# Autodesk Inventor assembly: magnet_ring_assembly
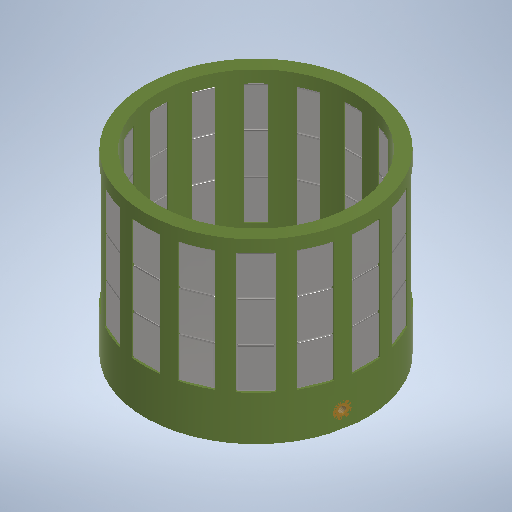
[picture p0: Inventor's stored thumbnail of the model, 512x512]
Saved by Autodesk Inventor 2025 (Build 290162000, 162)
## iProperties
Created: 2026-08-03
Part Number: magnet_ring_assembly
Document SubType Name: Assembly
Designer: zzapa
Author: zzapa
## Documents named in this file (4)
- C:\Users\zzapa\Desktop\Projekty\elektronika\engine-project\model\assemblies\magnet_ring_assembly.iam
- C:\Users\zzapa\Desktop\Projekty\elektronika\engine-project\model\parts\magnet_ring.ipt
- C:\Users\zzapa\Desktop\Projekty\elektronika\engine-project\model\parts\stator_magnet.ipt
- C:\Users\zzapa\Documents\Inventor\Content Center Files\R2025\pl-PL\GB 809-88 A\Nut GB 809 A M2 x 3.ipt
## Components (51 placed, 3 different names)
1. magnet_ring:1 — Zestawiające:1, Kątowe:1, Zestawiające:6, Równoległe:5, Zestawiające:7, Zestawiające:8, Równoległe:7, Zestawiające:9, Równoległe:8
2. Nut GB/T 809-1988 Type A M2x3:1 — Zestawiające:8, Równoległe:7
3. Nut GB/T 809-1988 Type A M2x3:2 — Zestawiające:9, Równoległe:8
4. stator_magnet:1 — Zestawiające:3, Równoległe:1, Równoległe:2, Zestawiające:6, Symetria:1, Symetria:2
5. stator_magnet:2 — Zestawiające:4, Równoległe:3, Równoległe:4, Symetria:1
6. stator_magnet:3 — Zestawiające:3, Równoległe:1, Zestawiające:4, Równoległe:2, Równoległe:3, Równoległe:4, Zestawiające:7, Symetria:2
7. stator_magnet:4
8. stator_magnet:5
9. stator_magnet:6
10. stator_magnet:7
11. stator_magnet:8
12. stator_magnet:9
13. stator_magnet:10
14. stator_magnet:11
15. stator_magnet:12
16. stator_magnet:13
17. stator_magnet:14
18. stator_magnet:15
19. stator_magnet:16
20. stator_magnet:17
21. stator_magnet:18
22. stator_magnet:19
23. stator_magnet:20
24. stator_magnet:21
25. stator_magnet:22
26. stator_magnet:23
27. stator_magnet:24 — Symetria:3
28. stator_magnet:25
29. stator_magnet:26
30. stator_magnet:27 — Symetria:3
31. stator_magnet:28
32. stator_magnet:29
33. stator_magnet:30
34. stator_magnet:31
35. stator_magnet:32
36. stator_magnet:33
37. stator_magnet:34
38. stator_magnet:35
39. stator_magnet:36
40. stator_magnet:37
41. stator_magnet:38
42. stator_magnet:39
43. stator_magnet:40
44. stator_magnet:41
45. stator_magnet:42
46. stator_magnet:43
47. stator_magnet:44
48. stator_magnet:45
49. stator_magnet:46
50. stator_magnet:47
51. stator_magnet:48
## Component patterns: (16 elements, first: stator_magnet:1 + stator_magnet:2 + stator_magnet:3)
## Relationships (19: Flush 8, Mate 7, Symmetry 3, Angle 1)
- Zestawiające:1 [Mate]: magnet_ring:1
- Kątowe:1 [Angle] (0 deg): magnet_ring:1
- Zestawiające:3 [Mate]: stator_magnet:1 ↔ stator_magnet:3
- Równoległe:1 [Flush]: stator_magnet:1 ↔ stator_magnet:3
- Zestawiające:4 [Mate]: stator_magnet:2 ↔ stator_magnet:3
- Równoległe:2 [Flush]: stator_magnet:1 ↔ stator_magnet:3
- Równoległe:3 [Flush]: stator_magnet:2 ↔ stator_magnet:3
- Równoległe:4 [Flush]: stator_magnet:2 ↔ stator_magnet:3
- Zestawiające:6 [Mate]: magnet_ring:1 ↔ stator_magnet:1
- Symetria:1 [Symmetry]: stator_magnet:1 ↔ stator_magnet:2
- Równoległe:5 [Flush]: magnet_ring:1
- Zestawiające:7 [Mate]: magnet_ring:1 ↔ stator_magnet:3
- Symetria:2 [Symmetry]: stator_magnet:1 ↔ stator_magnet:3
- Równoległe:6 [Flush]
- Symetria:3 [Symmetry]: stator_magnet:24 ↔ stator_magnet:27
- Zestawiające:8 [Mate]: magnet_ring:1 ↔ Nut GB/T 809-1988 Type A M2x3:1
- Równoległe:7 [Flush]: magnet_ring:1 ↔ Nut GB/T 809-1988 Type A M2x3:1
- Zestawiające:9 [Mate]: magnet_ring:1 ↔ Nut GB/T 809-1988 Type A M2x3:2
- Równoległe:8 [Flush]: magnet_ring:1 ↔ Nut GB/T 809-1988 Type A M2x3:2
